# Autodesk Inventor assembly: main_assembly
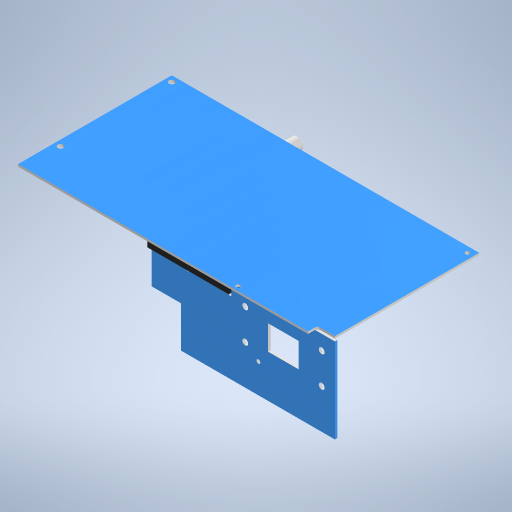
[picture p0: Inventor's stored thumbnail of the model, 512x512]
Saved by Autodesk Inventor 2024 (Build 280153000, 153)
## iProperties
Created: 2024-09-23
Part Number: main_assembly
Document SubType Name: Assembly
Designer: PC
Author: PC
## Documents named in this file (3)
- C:\Users\PC\Desktop\fotolito_czesci\main_assembly.iam
- C:\Users\PC\Desktop\fotolito_czesci\daughterboard.ipt
- C:\Users\PC\Desktop\fotolito_czesci\motherboard.ipt
## Components (2 placed, 2 different names)
1. daughterboard:1 — Mate:1, Mate:2, Mate:3
2. motherboard:1 — Mate:1, Mate:2, Mate:3
## Relationships (3: Mate 3)
- Mate:1: daughterboard:1 ↔ motherboard:1
- Mate:2: daughterboard:1 ↔ motherboard:1
- Mate:3 (1.75 mm): daughterboard:1 ↔ motherboard:1
